# Autodesk Inventor assembly: Front bar with Motors
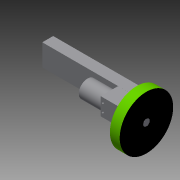
[picture p0: Inventor's stored thumbnail of the model, 180x180]
Saved by Autodesk Inventor 2015 (Build 190159000, 159)
## iProperties
Created: 2015-01-21
Part Number: Front bar with Motors
Document SubType Name: Assembly
Designer: chapale16
Author: chapale16
## Documents named in this file (4)
- \\lhssvr02\Homedirs\Robotics Club\CAD Model 2015\Front bar with Motors.iam
- \\lhssvr02\Homedirs\Robotics Club\CAD Model 2015\Modified Front Frame 27 in.ipt
- \\lhssvr02\Homedirs\Robotics Club\CAD Model 2015\Game Components\The Tote Collector-Arms\P60 Gear Box.ipt
- \\lhssvr02\Homedirs\Robotics Club\CAD Model 2015\Game Components\The Tote Collector-Arms\collector arm wheel.ipt
## Components (3 placed, 3 different names)
1. Modified Front Frame 27 in:1 — Mate:6, Flush:6, Flush:7, Flush:9
2. P60 Gear Box:1 — Mate:5, Mate:6, Flush:6, Flush:7, Flush:8, Flush:9
3. collector arm wheel:2 — Mate:5, Flush:8
## Relationships (6: Flush 4, Mate 2)
- Mate:5: P60 Gear Box:1 ↔ collector arm wheel:2
- Mate:6: Modified Front Frame 27 in:1 ↔ P60 Gear Box:1
- Flush:6: Modified Front Frame 27 in:1 ↔ P60 Gear Box:1
- Flush:7 (6.35 mm): Modified Front Frame 27 in:1 ↔ P60 Gear Box:1
- Flush:8: P60 Gear Box:1 ↔ collector arm wheel:2
- Flush:9: Modified Front Frame 27 in:1 ↔ P60 Gear Box:1
